# Autodesk Inventor assembly: full_assy
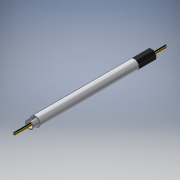
[picture p0: Inventor's stored thumbnail of the model, 180x180]
Saved by Autodesk Inventor 2017 (Build 210142000, 142)
## iProperties
Created: 2018-11-30
Part Number: full_assy
Document SubType Name: Assembly
Designer: ddeboer
Author: ddeboer
## Documents named in this file (5)
- C:\Users\ddeboer\Desktop\sch40_conduit\full_assy.iam
- C:\Users\ddeboer\Desktop\sch40_conduit\outer_assy.iam
- C:\Users\ddeboer\Desktop\sch40_conduit\inner_assy.iam
- C:\Users\ddeboer\Desktop\sch40_conduit\insert.ipt
- C:\Users\ddeboer\Desktop\sch40_conduit\cables.ipt
## Components (4 placed, 4 different names)
1. outer_assy:1 [sub-assembly] — Insert:1
2. inner_assy:1 [sub-assembly] — Insert:1, Insert:2, Mate:1, Insert:3
3. insert:1 — Insert:2, Mate:1
4. cables:1 — Insert:3
## Relationships (4: Insert 3, Mate 1)
- Insert:1: outer_assy:1 ↔ inner_assy:1
- Insert:2: inner_assy:1 ↔ insert:1
- Mate:1: inner_assy:1 ↔ insert:1
- Insert:3 (-60 mm): inner_assy:1 ↔ cables:1
